# Autodesk Inventor assembly: DRILL_JIG_Assembly1
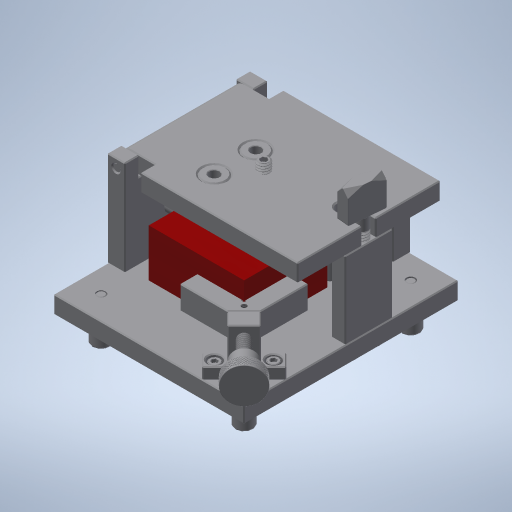
[picture p0: Inventor's stored thumbnail of the model, 512x512]
Saved by Autodesk Inventor 2024 (Build 280153000, 153)
## iProperties
Created: 2024-12-11
Part Number: DRILL_JIG_Assembly1
Document SubType Name: Assembly
Designer: NK
Author: NK
## Documents named in this file (20)
- D:\INVENTOR\CAD3135\100918925\ACITVITY_12\DRILL_JIG_Assembly1.iam
- D:\INVENTOR\CAD3135\100918925\ACITVITY_12\activity_12\base.ipt
- D:\INVENTOR\CAD3135\100918925\ACITVITY_12\activity_12\Plate_1.ipt
- D:\INVENTOR\CAD3135\100918925\ACITVITY_12\activity_12\Plate_2.ipt
- D:\INVENTOR\CAD3135\100918925\ACITVITY_12\activity_12\Plate_3.ipt
- D:\INVENTOR\CAD3135\100918925\ACITVITY_12\activity_12\Plate_4.ipt
- D:\INVENTOR\CAD3135\100918925\ACITVITY_12\activity_12\98381A487_Dowel Pin\98381A487_Dowel Pin.ipt
- D:\INVENTOR\CAD3135\100918925\ACITVITY_12\activity_12\91251A157_Black-Oxide Alloy Steel Socket Head Screw\91251A157_Black-Oxide Alloy Steel Socket Head Screw.ipt
- D:\INVENTOR\CAD3135\100918925\ACITVITY_12\activity_12\91251A158_Black-Oxide Alloy Steel Socket Head Screw\91251A158_Black-Oxide Alloy Steel Socket Head Screw.ipt
- D:\INVENTOR\CAD3135\100918925\ACITVITY_12\activity_12\91864A023_Black-Oxide Alloy Steel Socket Head Screw\91864A023_Black-Oxide Alloy Steel Socket Head Screw.ipt
- D:\INVENTOR\CAD3135\100918925\ACITVITY_12\activity_12\8511A23_Press-Fit Locating and Support Button\8511A23_Press-Fit Locating and Support Button.ipt
- D:\INVENTOR\CAD3135\100918925\ACITVITY_12\activity_12\8511A415_Press-Fit Locating and Support Button\8511A415_Press-Fit Locating and Support Button.ipt
- D:\INVENTOR\CAD3135\100918925\ACITVITY_12\activity_12\Riser_Block.ipt
- D:\INVENTOR\CAD3135\100918925\ACITVITY_12\activity_12\98381A626_Dowel Pin (1)\98381A626_Dowel Pin (1).ipt
- D:\INVENTOR\CAD3135\100918925\ACITVITY_12\activity_12\Corner_Clamp.ipt
- D:\INVENTOR\CAD3135\100918925\ACITVITY_12\activity_12\6079K14_Black-Oxide Steel Knurled Grip Knob.ipt
- D:\INVENTOR\CAD3135\100918925\ACITVITY_12\activity_12\Leaf.ipt
- D:\INVENTOR\CAD3135\100918925\ACITVITY_12\activity_12\8491A247_Press-Fit Drill Bushing\8491A247_Press-Fit Drill Bushing.ipt
- D:\INVENTOR\CAD3135\100918925\ACITVITY_12\activity_12\90017A547_Latching Thumb Screw\90017A547_Latching Thumb Screw.ipt
- D:\INVENTOR\CAD3135\100918925\ACITVITY_12\activity_12\92432A456_Swivel-Tip Set Screw\92432A456_Swivel-Tip Set Screw.ipt
## Components (35 placed, 19 different names)
1. base:1 — Insert:1, Insert:2, Insert:3, Insert:4, Insert:5, Insert:6, Insert:7, Insert:8, Insert:9, Insert:10, Insert:13, Insert:14, Insert:17, Insert:18, Insert:19, Insert:20, Insert:24, Insert:25, Insert:26, Insert:27, Insert:28, Insert:29, Insert:30
2. Plate_1:1 — Insert:1, Insert:2, Insert:11, Insert:12, Insert:21
3. Plate_2:1 — Insert:3, Insert:4, Insert:22, Insert:23, Insert:33, Insert:36, Insert:37
4. Plate_3:1 — Insert:5, Insert:6, Mate:1, Insert:38
5. Plate_4:1 — Insert:7, Insert:8, Insert:15, Insert:16, Insert:31, Insert:32
6. 98381A487_Dowel Pin:1 — Insert:10
7. 98381A487_Dowel Pin:2 — Insert:9
8. 91251A157_Black-Oxide Alloy Steel Socket Head Screw:1 — Insert:12
9. 91251A157_Black-Oxide Alloy Steel Socket Head Screw:2 — Insert:11
10. 91251A158_Black-Oxide Alloy Steel Socket Head Screw:1 — Insert:13
11. 91251A158_Black-Oxide Alloy Steel Socket Head Screw:2 — Insert:14
12. 91864A023_Black-Oxide Alloy Steel Socket Head Screw:1 — Insert:15
13. 91864A023_Black-Oxide Alloy Steel Socket Head Screw:2 — Insert:16
14. 8511A23_Press-Fit Locating and Support Button:1 — Insert:17
15. 8511A23_Press-Fit Locating and Support Button:2 — Insert:18
16. 8511A23_Press-Fit Locating and Support Button:3 — Insert:19
17. 8511A23_Press-Fit Locating and Support Button:4 — Insert:20
18. 8511A415_Press-Fit Locating and Support Button:1 — Insert:21
19. 8511A415_Press-Fit Locating and Support Button:2 — Insert:22
20. 8511A415_Press-Fit Locating and Support Button:3 — Insert:23
21. 8511A415_Press-Fit Locating and Support Button:4 — Insert:26
22. 8511A415_Press-Fit Locating and Support Button:5 — Insert:24
23. 8511A415_Press-Fit Locating and Support Button:6 — Insert:25
24. 8511A415_Press-Fit Locating and Support Button:7 — Insert:27
25. Riser_Block:1 — Insert:28, Insert:29
26. 98381A626_Dowel Pin (1):1 — Insert:30
27. Corner_Clamp:1 — Insert:31
28. 6079K14_Black-Oxide Steel Knurled Grip Knob:1 — Insert:32
29. Leaf:1 — Insert:33, Mate:1, Insert:34, Insert:35, Insert:39
30. 8491A247_Press-Fit Drill Bushing:1 — Insert:35
31. 8491A247_Press-Fit Drill Bushing:2 — Insert:34
32. 98381A487_Dowel Pin:3 — Insert:36
33. 98381A487_Dowel Pin:4 — Insert:37
34. 90017A547_Latching Thumb Screw:1 — Insert:38
35. 92432A456_Swivel-Tip Set Screw:1 — Insert:39
## Relationships (40: Insert 39, Mate 1)
- Insert:1: base:1 ↔ Plate_1:1
- Insert:2: base:1 ↔ Plate_1:1
- Insert:3: base:1 ↔ Plate_2:1
- Insert:4: base:1 ↔ Plate_2:1
- Insert:5: base:1 ↔ Plate_3:1
- Insert:6: base:1 ↔ Plate_3:1
- Insert:7: base:1 ↔ Plate_4:1
- Insert:8: base:1 ↔ Plate_4:1
- Insert:9: base:1 ↔ 98381A487_Dowel Pin:2
- Insert:10: base:1 ↔ 98381A487_Dowel Pin:1
- Insert:11 (-43.18 mm): Plate_1:1 ↔ 91251A157_Black-Oxide Alloy Steel Socket Head Screw:2
- Insert:12 (-43.18 mm): Plate_1:1 ↔ 91251A157_Black-Oxide Alloy Steel Socket Head Screw:1
- Insert:13 (-43.18 mm): base:1 ↔ 91251A158_Black-Oxide Alloy Steel Socket Head Screw:1
- Insert:14 (-43.18 mm): base:1 ↔ 91251A158_Black-Oxide Alloy Steel Socket Head Screw:2
- Insert:15: Plate_4:1 ↔ 91864A023_Black-Oxide Alloy Steel Socket Head Screw:1
- Insert:16: Plate_4:1 ↔ 91864A023_Black-Oxide Alloy Steel Socket Head Screw:2
- Insert:17: base:1 ↔ 8511A23_Press-Fit Locating and Support Button:1
- Insert:18: base:1 ↔ 8511A23_Press-Fit Locating and Support Button:2
- Insert:19: base:1 ↔ 8511A23_Press-Fit Locating and Support Button:3
- Insert:20: base:1 ↔ 8511A23_Press-Fit Locating and Support Button:4
- Insert:21: Plate_1:1 ↔ 8511A415_Press-Fit Locating and Support Button:1
- Insert:22: Plate_2:1 ↔ 8511A415_Press-Fit Locating and Support Button:2
- Insert:23: Plate_2:1 ↔ 8511A415_Press-Fit Locating and Support Button:3
- Insert:24: base:1 ↔ 8511A415_Press-Fit Locating and Support Button:5
- Insert:25: base:1 ↔ 8511A415_Press-Fit Locating and Support Button:6
- Insert:26: base:1 ↔ 8511A415_Press-Fit Locating and Support Button:4
- Insert:27: base:1 ↔ 8511A415_Press-Fit Locating and Support Button:7
- Insert:28: base:1 ↔ Riser_Block:1
- Insert:29: base:1 ↔ Riser_Block:1
- Insert:30: base:1 ↔ 98381A626_Dowel Pin (1):1
- Insert:31: Plate_4:1 ↔ Corner_Clamp:1
- Insert:32 (-7.62 mm): Plate_4:1 ↔ 6079K14_Black-Oxide Steel Knurled Grip Knob:1
- Insert:33: Plate_2:1 ↔ Leaf:1
- Mate:1: Plate_3:1 ↔ Leaf:1
- Insert:34: Leaf:1 ↔ 8491A247_Press-Fit Drill Bushing:2
- Insert:35: Leaf:1 ↔ 8491A247_Press-Fit Drill Bushing:1
- Insert:36: Plate_2:1 ↔ 98381A487_Dowel Pin:3
- Insert:37: Plate_2:1 ↔ 98381A487_Dowel Pin:4
- Insert:38 (-20.32 mm): Plate_3:1 ↔ 90017A547_Latching Thumb Screw:1
- Insert:39: Leaf:1 ↔ 92432A456_Swivel-Tip Set Screw:1
